# Autodesk Inventor assembly: c7697-la-015_v0-13
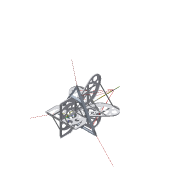
[picture p0: Inventor's stored thumbnail of the model, 180x180]
Saved by Autodesk Inventor 2019.3 (Build 233278000, 278)
## iProperties
Created: 2018-08-09
Part Number: c7697-la-015_v0-13
Document SubType Name: Assembly
Designer: Kathryn Rosie
Sending System: CREO PARAMETRIC BY PTC INC, 2017170
Preprocessor: CREO PARAMETRIC BY PTC INC, 2017170
Title: C7697-LA-015_ASM
Author: namd
Revision Number: 1LAST_VERSION
## Documents named in this file (24)
- C:\Users\Kathryn Rosie\Google Drive\HERA\Feed\Feed CAD\c7697-la-015_v0-13.iam
- C:\Users\Kathryn Rosie\Google Drive\HERA\Feed\Feed CAD\C7697-SA-019_ASM.iam
- C:\Users\Kathryn Rosie\Google Drive\HERA\Feed\Feed CAD\C7697-SA-017_ASM.iam
- C:\Users\Kathryn Rosie\Google Drive\HERA\Feed\Feed CAD\C7697-SK-164.ipt
- C:\Users\Kathryn Rosie\Google Drive\HERA\Feed\Feed CAD\C7697-SK-155.ipt
- C:\Users\Kathryn Rosie\Google Drive\HERA\Feed\Feed CAD\C7697-DP-127.ipt
- C:\Users\Kathryn Rosie\Google Drive\HERA\Feed\Feed CAD\C7697-SK-151.ipt
- C:\Users\Kathryn Rosie\Google Drive\HERA\Feed\Feed CAD\C7697-DP-111.ipt
- C:\Users\Kathryn Rosie\Google Drive\HERA\Feed\Feed CAD\C7697-DP-112.ipt
- C:\Users\Kathryn Rosie\Google Drive\HERA\Feed\Feed CAD\C7697-SK-149.ipt
- C:\Users\Kathryn Rosie\Google Drive\HERA\Feed\Feed CAD\C7697-DP-114.ipt
- C:\Users\Kathryn Rosie\Google Drive\HERA\Feed\Feed CAD\C7697-SK-174.ipt
- C:\Users\Kathryn Rosie\Google Drive\HERA\Feed\Feed CAD\C7697-SA-022_ASM.iam
- C:\Users\Kathryn Rosie\Google Drive\HERA\Feed\Feed CAD\C7697-SK-167.ipt
- C:\Users\Kathryn Rosie\Google Drive\HERA\Feed\Feed CAD\C7697-DP-130.ipt
- C:\Users\Kathryn Rosie\Google Drive\HERA\Feed\Feed CAD\C7697-SK-142.ipt
- C:\Users\Kathryn Rosie\Google Drive\HERA\Feed\Feed CAD\C7697-SK-145.ipt
- C:\Users\Kathryn Rosie\Google Drive\HERA\Feed\Feed CAD\C7697-SK-148.ipt
- C:\Users\Kathryn Rosie\Google Drive\HERA\Feed\Feed CAD\C7697-SK-143.ipt
- C:\Users\Kathryn Rosie\Google Drive\HERA\Feed\Feed CAD\C7697-SK-141.ipt
- C:\Users\Kathryn Rosie\Google Drive\HERA\Feed\Feed CAD\C7697-SK-146.ipt
- C:\Users\Kathryn Rosie\Google Drive\HERA\Feed\Feed CAD\Conduit-brace.ipt
- C:\Users\Kathryn Rosie\Google Drive\HERA\Feed\Feed CAD\C7697-DP-113_v0.10.ipt
- C:\Users\Kathryn Rosie\Google Drive\HERA\Feed\Feed CAD\SA-117_v0.2.iam
## Components (198 placed, 197 different names)
1. 114 [sub-assembly] — Mate:8, Mate:9, Mate:11, Mate:12, Mate:13, Angle:1, Mate:16, Mate:25, Mate:26, Mate:27, Mate:66, Mate:67, Mate:68, Mate:79, Mate:81, Mate:83, Mate:85
2. 118 [sub-assembly] — Flush:3, Flush:4, Mate:73, Mate:100, Mate:103, Mate:105, Mate:106, Mate:111, Mate:112, Mate:116, Mate:122, Mate:123, Mate:124, Mate:139, Mate:232, Mate:233, Mate:234, Mate:235, Mate:236, Mate:237, Mate:238, Mate:239, Mate:240, Mate:290
3. 119 [sub-assembly] — Flush:3, Mate:89, Mate:90, Mate:91, Mate:92, Mate:93, Mate:117, Mate:121, Mate:131, Mate:132, Mate:133, Mate:244, Mate:245, Mate:246, Mate:247, Mate:248, Mate:249, Mate:250, Mate:251, Mate:252, Mate:303
4. 120 [sub-assembly] — Mate:44, Mate:45, Mate:46, Mate:97, Mate:108, Mate:109, Mate:114, Mate:115, Mate:128, Mate:130, Mate:147, Mate:148, Mate:149, Mate:194, Mate:256, Mate:257, Mate:258, Mate:259, Mate:260, Mate:261, Mate:262, Mate:263, Mate:264
5. 121 [sub-assembly] — Flush:4, Mate:8, Mate:15, Mate:51, Mate:52, Mate:53, Mate:98, Mate:99, Mate:102, Mate:110, Mate:125, Mate:126, Mate:127, Mate:223, Mate:224, Mate:225, Mate:226, Mate:227, Mate:228, Mate:268, Mate:269, Mate:270
6. 122 — Mate:237, Mate:238, Mate:241
7. 123 — Mate:236, Mate:239, Mate:242
8. 124 — Mate:235, Mate:240, Mate:243
9. 125 — Mate:241, Mate:246
10. 126 — Mate:242, Mate:245
11. 127 — Mate:243, Mate:244
12. 128 — Mate:247, Mate:252, Mate:255
13. 129 — Mate:248, Mate:251, Mate:254
14. 130 — Mate:249, Mate:250, Mate:253
15. 131 — Mate:255, Mate:256
16. 132 — Mate:254, Mate:257
17. 133 — Mate:253, Mate:258
18. 134 — Mate:259, Mate:264, Mate:267
19. 135 — Mate:260, Mate:263, Mate:266
20. 136 — Mate:261, Mate:262, Mate:265
21. 137 — Mate:267, Mate:268
22. 138 — Mate:266, Mate:269
23. 139 — Mate:265, Mate:270
24. 140 — Mate:225, Mate:226, Mate:229
25. 141 — Mate:224, Mate:227, Mate:230
26. 142 — Mate:223, Mate:228, Mate:231
27. 143 — Mate:229, Mate:232
28. 144 — Mate:230, Mate:233
29. 145 — Mate:231, Mate:234
30. 146 — Mate:69, Mate:70, Angle:4, Mate:71, Mate:72
31. 147 — Mate:87, Mate:88, Angle:5, Mate:93, Mate:94
32. 148 — Mate:21, Mate:22, Angle:2, Mate:42, Mate:43, Mate:45
33. 149 — Mate:47, Angle:3, Mate:48, Mate:49, Mate:50, Mate:52
34. 150 — Mate:71, Mate:73
35. 151 — Mate:72
36. 152 — Mate:89, Mate:91, Mate:94
37. 153 — Mate:90, Mate:92
38. 154 — Mate:42, Mate:44, Mate:46
39. 155 — Mate:43
40. 156 — Mate:49, Mate:51
41. 157 — Mate:50, Mate:53
42. 158 — Mate:99, Mate:100, Mate:103, Mate:158, Mate:159, Mate:160, Mate:161, Mate:162, Mate:163, Mate:164, Mate:165, Mate:174, Mate:175, Mate:176, Mate:177, Mate:186, Mate:187, Mate:188, Mate:189
43. 159 — Mate:105, Mate:106, Mate:133, Mate:170, Mate:171, Mate:172, Mate:173, Mate:213, Mate:215, Mate:216, Mate:217, Mate:218, Mate:219
44. 160 — Mate:108, Mate:109, Mate:195, Mate:196, Mate:197, Mate:198, Mate:199, Mate:212, Mate:214, Mate:220, Mate:221, Mate:222
45. 161 — Mate:97, Mate:98, Mate:102, Mate:178, Mate:179, Mate:180, Mate:181, Mate:190, Mate:191, Mate:192, Mate:193, Mate:194, Mate:204, Mate:205, Mate:206, Mate:207
46. 162 — Mate:38, Mate:40, Mate:67, Mate:84, Mate:86, Mate:277, Mate:279, Mate:281, Mate:283, Mate:284, Mate:285, Mate:286, Mate:287, Mate:288, Mate:289
47. 163 — Mate:36, Mate:37, Mate:66, Mate:80, Mate:82, Mate:290, Mate:294, Mate:295, Mate:296, Mate:297, Mate:298, Mate:299, Mate:300, Mate:301, Mate:302
48. 164 — Mate:25, Mate:31, Mate:32, Mate:77, Mate:78, Mate:303, Mate:307, Mate:308, Mate:309, Mate:310, Mate:311, Mate:312, Mate:313, Mate:314, Mate:315
49. 165 — Mate:11, Tangent:3, Tangent:4, Angle:1, Mate:14, Mate:15, Mate:33, Mate:34, Mate:68, Mate:75, Mate:76, Mate:271, Mate:272, Mate:273, Mate:274, Mate:275, Mate:276
50. 166 — Mate:27, Mate:78
51. 167 — Mate:26, Mate:77
52. 168
53. 169
54. 170 — Mate:13, Tangent:3, Mate:76
55. 171 — Mate:12, Tangent:4, Mate:75
56. 172
57. 173
58. 174 — Mate:85, Mate:86
59. 175 — Mate:83, Mate:84
60. 176
61. 177
62. 178 — Mate:81, Mate:82
63. 179 — Mate:79, Mate:80
64. 180
65. 181
66. 182 — Mate:110, Mate:111, Mate:112, Mate:145, Flush:8
67. 183 — Mate:116, Mate:117, Mate:139
68. 184 — Mate:130, Mate:131, Mate:132, Mate:143, Flush:7
69. 185 — Mate:114, Mate:115
70. 186 — Mate:124, Mate:125, Mate:126
71. 187 — Mate:121, Mate:122, Mate:123, Mate:151
72. 188 — Mate:148, Mate:149, Mate:150, Mate:153, Mate:154, Mate:155, Mate:156, Mate:157
73. 189 — Mate:127, Mate:128, Mate:129
74. 190 — Mate:162, Mate:163, Mate:168
75. 191 — Mate:161, Mate:164, Mate:167
76. 192 — Mate:160, Mate:165, Mate:166
77. 193 — Mate:158, Mate:159, Mate:169
78. 194 — Mate:284, Mate:287, Mate:293
79. 195 — Mate:285, Mate:288, Mate:292
80. 196 — Mate:286, Mate:289, Mate:291
81. 197
82. 198
83. 199
84. 200
85. 201
86. 202
87. 203 — Mate:168, Mate:172
88. 204 — Mate:167, Mate:173
89. 205 — Mate:166, Mate:171
90. 206 — Mate:169, Mate:170
91. 207 — Mate:293, Mate:296
92. 208 — Mate:292, Mate:295
93. 209 — Mate:291, Mate:294
94. 210
95. 211
96. 212
97. 213
98. 214
99. 215
100. 216 — Mate:211, Mate:212, Mate:213
101. 217 — Mate:210, Mate:217, Mate:218
102. 218 — Mate:209, Mate:216, Mate:219
103. 219 — Mate:208, Mate:215
104. 220 — Mate:297, Mate:300, Mate:306
105. 221 — Mate:298, Mate:301, Mate:305
106. 222 — Mate:299, Mate:302, Mate:304
107. 223
108. 224
109. 225
110. 226
111. 227 — Mate:150, Mate:151, Mate:152
112. 228
113. 229 — Mate:211, Mate:214
114. 230 — Mate:210, Mate:222
115. 231 — Mate:209, Mate:221
116. 232 — Mate:208, Mate:220
117. 233 — Mate:306, Mate:307
118. 234 — Mate:305, Mate:308
119. 235 — Mate:304, Mate:309
120. 236
121. 237
122. 238
123. 239
124. 240 — Mate:152, Mate:153
125. 241
126. 242 — Mate:190, Mate:196, Mate:203
127. 243 — Mate:191, Mate:195, Mate:197, Mate:202
128. 244 — Mate:192, Mate:198, Mate:201
129. 245 — Mate:193, Mate:199, Mate:200
130. 246 — Mate:310, Mate:313
131. 247 — Mate:311, Mate:314
132. 248 — Mate:312, Mate:315
133. 249
134. 250
135. 251
136. 252
137. 253 — Mate:147, Mate:154, Mate:155
138. 254 — Mate:129, Mate:156, Mate:157
139. 255 — Mate:203, Mate:207
140. 256 — Mate:202, Mate:206
141. 257 — Mate:201, Mate:205
142. 258 — Mate:200, Mate:204
143. 259
144. 260
145. 261
146. 262
147. 263
148. 264
149. 265
150. 266
151. 267
152. 268 — Mate:177, Mate:178, Mate:185
153. 269 — Mate:176, Mate:179, Mate:184
154. 270 — Mate:175, Mate:180, Mate:183
155. 271 — Mate:174, Mate:181, Mate:182
156. 272 — Mate:271, Mate:274, Mate:282
157. 273 — Mate:272, Mate:275, Mate:280
158. 274 — Mate:273, Mate:276, Mate:277, Mate:278
159. 275
160. 276
161. 277
162. 278
163. 279
164. 280
165. 281 — Mate:185, Mate:189
166. 282 — Mate:184, Mate:188
167. 283 — Mate:183, Mate:187
168. 284 — Mate:182, Mate:186
169. 285 — Mate:282, Mate:283
170. 286 — Mate:280, Mate:281
171. 287 — Mate:278, Mate:279
172. 288
173. 289
174. 290
175. 291
176. 292
177. 293
178. 305 [sub-assembly] — Mate:9, Mate:10, Mate:14, Mate:29, Mate:30, Mate:31, Mate:35, Mate:39, Mate:41, Mate:316
179. 306 — Mate:38, Mate:40, Mate:41
180. 307 — Mate:36, Mate:37, Mate:39
181. 308 — Mate:30, Mate:32
182. 309 — Mate:33, Mate:34, Mate:35
183. 310 — Mate:10
184. 311
185. 312
186. 313 — Mate:16, Mate:21, Mate:22, Angle:2, Mate:29, Mate:47, Angle:3, Mate:48, Mate:54, Mate:55, Mate:56, Mate:57, Mate:58, Mate:59, Mate:60, Mate:61, Mate:62, Mate:63, Mate:64, Mate:65, Mate:69, Mate:70, Angle:4, Mate:87, Mate:88, Angle:5
187. 314 — Mate:54, Mate:55
188. 315 — Mate:57, Mate:60
189. 316 — Mate:58, Mate:61
190. 317 — Mate:62, Mate:64
191. 318 — Mate:63, Mate:65
192. 319 — Mate:56, Mate:59
193. 320
194. 321
195. 346
196. Conduit-brace:1 — Mate:143, Flush:7, Mate:317, Angle:6
197. Conduit-brace:2 — Mate:145, Flush:8
198. SA-117_v0.2:1 [sub-assembly] — Mate:316, Mate:317, Angle:6
## Relationships (295: Mate 283, Angle 6, Flush 4, Tangent 2)
- Flush:3: 118 ↔ 119
- Flush:4: 118 ↔ 121
- Mate:8: 114 ↔ 121
- Mate:9: 114 ↔ 305
- Mate:10: 305 ↔ 310
- Mate:11: 114 ↔ 165
- Mate:12: 114 ↔ 171
- Mate:13: 114 ↔ 170
- Tangent:3: 165 ↔ 170
- Tangent:4: 165 ↔ 171
- Angle:1 (0 deg): 114 ↔ 165
- Mate:14: 165 ↔ 305
- Mate:15: 121 ↔ 165
- Mate:16: 114 ↔ 313
- Mate:21: 148 ↔ 313
- Mate:22: 148 ↔ 313
- Mate:25: 114 ↔ 164
- Mate:26: 114 ↔ 167
- Mate:27: 114 ↔ 166
- Angle:2 (180 deg): 148 ↔ 313
- Mate:29: 305 ↔ 313
- Mate:30: 305 ↔ 308
- Mate:31: 164 ↔ 305
- Mate:32: 164 ↔ 308
- Mate:33: 165 ↔ 309
- Mate:34: 165 ↔ 309
- Mate:35: 305 ↔ 309
- Mate:36: 163 ↔ 307
- Mate:37: 163 ↔ 307
- Mate:38: 162 ↔ 306
- Mate:39: 305 ↔ 307
- Mate:40: 162 ↔ 306
- Mate:41: 305 ↔ 306
- Mate:42: 148 ↔ 154
- Mate:43: 148 ↔ 155
- Mate:44: 120 ↔ 154
- Mate:45: 120 ↔ 148
- Mate:46: 120 ↔ 154
- Mate:47: 149 ↔ 313
- Angle:3 (180 deg): 149 ↔ 313
- Mate:48: 149 ↔ 313
- Mate:49: 149 ↔ 156
- Mate:50: 149 ↔ 157
- Mate:51: 121 ↔ 156
- Mate:52: 121 ↔ 149
- Mate:53: 121 ↔ 157
- Mate:54: 313 ↔ 314
- Mate:55: 313 ↔ 314
- Mate:56: 313 ↔ 319
- Mate:57: 313 ↔ 315
- Mate:58: 313 ↔ 316
- Mate:59: 313 ↔ 319
- Mate:60: 313 ↔ 315
- Mate:61: 313 ↔ 316
- Mate:62: 313 ↔ 317
- Mate:63: 313 ↔ 318
- Mate:64: 313 ↔ 317
- Mate:65: 313 ↔ 318
- Mate:66: 114 ↔ 163
- Mate:67: 114 ↔ 162
- Mate:68: 114 ↔ 165
- Mate:69: 146 ↔ 313
- Mate:70: 146 ↔ 313
- Angle:4 (0 deg): 146 ↔ 313
- Mate:71: 146 ↔ 150
- Mate:72: 146 ↔ 151
- Mate:73: 118 ↔ 150
- Mate:75: 165 ↔ 171
- Mate:76: 165 ↔ 170
- Mate:77: 164 ↔ 167
- Mate:78: 164 ↔ 166
- Mate:79: 114 ↔ 179
- Mate:80: 163 ↔ 179
- Mate:81: 114 ↔ 178
- Mate:82: 163 ↔ 178
- Mate:83: 114 ↔ 175
- Mate:84: 162 ↔ 175
- Mate:85: 114 ↔ 174
- Mate:86: 162 ↔ 174
- Mate:87: 147 ↔ 313
- Mate:88: 147 ↔ 313
- Angle:5 (0 deg): 147 ↔ 313
- Mate:89: 119 ↔ 152
- Mate:90: 119 ↔ 153
- Mate:91: 119 ↔ 152
- Mate:92: 119 ↔ 153
- Mate:93: 119 ↔ 147
- Mate:94: 147 ↔ 152
- Mate:97: 120 ↔ 161
- Mate:98: 121 ↔ 161
- Mate:99: 121 ↔ 158
- Mate:100: 118 ↔ 158
- Mate:102: 121 ↔ 161
- Mate:103: 118 ↔ 158
- Mate:105: 118 ↔ 159
- Mate:106: 118 ↔ 159
- Mate:108: 120 ↔ 160
- Mate:109: 120 ↔ 160
- Mate:110: 121 ↔ 182
- Mate:111: 118 ↔ 182
- Mate:112: 118 ↔ 182
- Mate:114: 120 ↔ 185
- Mate:115: 120 ↔ 185
- Mate:116: 118 ↔ 183
- Mate:117: 119 ↔ 183
- Mate:121: 119 ↔ 187
- Mate:122: 118 ↔ 187
- Mate:123: 118 ↔ 187
- Mate:124: 118 ↔ 186
- Mate:125: 121 ↔ 186
- Mate:126: 121 ↔ 186
- Mate:127: 121 ↔ 189
- Mate:128: 120 ↔ 189
- Mate:129: 189 ↔ 254
- Mate:130: 120 ↔ 184
- Mate:131: 119 ↔ 184
- Mate:132: 119 ↔ 184
- Mate:133: 119 ↔ 159
- Mate:139: 118 ↔ 183
- Mate:143: 184 ↔ Conduit-brace:1
- Flush:7: 184 ↔ Conduit-brace:1
- Mate:145: 182 ↔ Conduit-brace:2
- Flush:8: 182 ↔ Conduit-brace:2
- Mate:147: 120 ↔ 253
- Mate:148: 120 ↔ 188
- Mate:149: 120 ↔ 188
- Mate:150: 188 ↔ 227
- Mate:151: 187 ↔ 227
- Mate:152: 227 ↔ 240
- Mate:153: 188 ↔ 240
- Mate:154: 188 ↔ 253
- Mate:155: 188 ↔ 253
- Mate:156: 188 ↔ 254
- Mate:157: 188 ↔ 254
- Mate:158: 158 ↔ 193
- Mate:159: 158 ↔ 193
- Mate:160: 158 ↔ 192
- Mate:161: 158 ↔ 191
- Mate:162: 158 ↔ 190
- Mate:163: 158 ↔ 190
- Mate:164: 158 ↔ 191
- Mate:165: 158 ↔ 192
- Mate:166: 192 ↔ 205
- Mate:167: 191 ↔ 204
- Mate:168: 190 ↔ 203
- Mate:169: 193 ↔ 206
- Mate:170: 159 ↔ 206
- Mate:171: 159 ↔ 205
- Mate:172: 159 ↔ 203
- Mate:173: 159 ↔ 204
- Mate:174: 158 ↔ 271
- Mate:175: 158 ↔ 270
- Mate:176: 158 ↔ 269
- Mate:177: 158 ↔ 268
- Mate:178: 161 ↔ 268
- Mate:179: 161 ↔ 269
- Mate:180: 161 ↔ 270
- Mate:181: 161 ↔ 271
- Mate:182: 271 ↔ 284
- Mate:183: 270 ↔ 283
- Mate:184: 269 ↔ 282
- Mate:185: 268 ↔ 281
- Mate:186: 158 ↔ 284
- Mate:187: 158 ↔ 283
- Mate:188: 158 ↔ 282
- Mate:189: 158 ↔ 281
- Mate:190: 161 ↔ 242
- Mate:191: 161 ↔ 243
- Mate:192: 161 ↔ 244
- Mate:193: 161 ↔ 245
- Mate:194: 120 ↔ 161
- Mate:195: 160 ↔ 243
- Mate:196: 160 ↔ 242
- Mate:197: 160 ↔ 243
- Mate:198: 160 ↔ 244
- Mate:199: 160 ↔ 245
- Mate:200: 245 ↔ 258
- Mate:201: 244 ↔ 257
- Mate:202: 243 ↔ 256
- Mate:203: 242 ↔ 255
- Mate:204: 161 ↔ 258
- Mate:205: 161 ↔ 257
- Mate:206: 161 ↔ 256
- Mate:207: 161 ↔ 255
- Mate:208: 219 ↔ 232
- Mate:209: 218 ↔ 231
- Mate:210: 217 ↔ 230
- Mate:211: 216 ↔ 229
- Mate:212: 160 ↔ 216
- Mate:213: 159 ↔ 216
- Mate:214: 160 ↔ 229
- Mate:215: 159 ↔ 219
- Mate:216: 159 ↔ 218
- Mate:217: 159 ↔ 217
- Mate:218: 159 ↔ 217
- Mate:219: 159 ↔ 218
- Mate:220: 160 ↔ 232
- Mate:221: 160 ↔ 231
- Mate:222: 160 ↔ 230
- Mate:223: 121 ↔ 142
- Mate:224: 121 ↔ 141
- Mate:225: 121 ↔ 140
- Mate:226: 121 ↔ 140
- Mate:227: 121 ↔ 141
- Mate:228: 121 ↔ 142
- Mate:229: 140 ↔ 143
- Mate:230: 141 ↔ 144
- Mate:231: 142 ↔ 145
- Mate:232: 118 ↔ 143
- Mate:233: 118 ↔ 144
- Mate:234: 118 ↔ 145
- Mate:235: 118 ↔ 124
- Mate:236: 118 ↔ 123
- Mate:237: 118 ↔ 122
- Mate:238: 118 ↔ 122
- Mate:239: 118 ↔ 123
- Mate:240: 118 ↔ 124
- Mate:241: 122 ↔ 125
- Mate:242: 123 ↔ 126
- Mate:243: 124 ↔ 127
- Mate:244: 119 ↔ 127
- Mate:245: 119 ↔ 126
- Mate:246: 119 ↔ 125
- Mate:247: 119 ↔ 128
- Mate:248: 119 ↔ 129
- Mate:249: 119 ↔ 130
- Mate:250: 119 ↔ 130
- Mate:251: 119 ↔ 129
- Mate:252: 119 ↔ 128
- Mate:253: 130 ↔ 133
- Mate:254: 129 ↔ 132
- Mate:255: 128 ↔ 131
- Mate:256: 120 ↔ 131
- Mate:257: 120 ↔ 132
- Mate:258: 120 ↔ 133
- Mate:259: 120 ↔ 134
- Mate:260: 120 ↔ 135
- Mate:261: 120 ↔ 136
- Mate:262: 120 ↔ 136
- Mate:263: 120 ↔ 135
- Mate:264: 120 ↔ 134
- Mate:265: 136 ↔ 139
- Mate:266: 135 ↔ 138
- Mate:267: 134 ↔ 137
- Mate:268: 121 ↔ 137
- Mate:269: 121 ↔ 138
- Mate:270: 121 ↔ 139
- Mate:271: 165 ↔ 272
- Mate:272: 165 ↔ 273
- Mate:273: 165 ↔ 274
- Mate:274: 165 ↔ 272
- Mate:275: 165 ↔ 273
- Mate:276: 165 ↔ 274
- Mate:277: 162 ↔ 274
- Mate:278: 274 ↔ 287
- Mate:279: 162 ↔ 287
- Mate:280: 273 ↔ 286
- Mate:281: 162 ↔ 286
- Mate:282: 272 ↔ 285
- Mate:283: 162 ↔ 285
- Mate:284: 162 ↔ 194
- Mate:285: 162 ↔ 195
- Mate:286: 162 ↔ 196
- Mate:287: 162 ↔ 194
- Mate:288: 162 ↔ 195
- Mate:289: 162 ↔ 196
- Mate:290: 118 ↔ 163
- Mate:291: 196 ↔ 209
- Mate:292: 195 ↔ 208
- Mate:293: 194 ↔ 207
- Mate:294: 163 ↔ 209
- Mate:295: 163 ↔ 208
- Mate:296: 163 ↔ 207
- Mate:297: 163 ↔ 220
- Mate:298: 163 ↔ 221
- Mate:299: 163 ↔ 222
- Mate:300: 163 ↔ 220
- Mate:301: 163 ↔ 221
- Mate:302: 163 ↔ 222
- Mate:303: 119 ↔ 164
- Mate:304: 222 ↔ 235
- Mate:305: 221 ↔ 234
- Mate:306: 220 ↔ 233
- Mate:307: 164 ↔ 233
- Mate:308: 164 ↔ 234
- Mate:309: 164 ↔ 235
- Mate:310: 164 ↔ 246
- Mate:311: 164 ↔ 247
- Mate:312: 164 ↔ 248
- Mate:313: 164 ↔ 246
- Mate:314: 164 ↔ 247
- Mate:315: 164 ↔ 248
- Mate:316: 305 ↔ SA-117_v0.2:1
- Mate:317: Conduit-brace:1 ↔ SA-117_v0.2:1
- Angle:6 (0 deg): Conduit-brace:1 ↔ SA-117_v0.2:1
